# Autodesk Inventor assembly: meccanum_wheel_base_norm
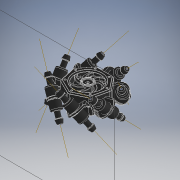
[picture p0: Inventor's stored thumbnail of the model, 180x180]
Saved by Autodesk Inventor 2022 (Build 260153000, 153)
## iProperties
Created: 2023-01-06
Part Number: meccanum_wheel_base_norm
Document SubType Name: Assembly
Designer: Иван Петров
Author: Иван Петров
## Documents named in this file (3)
- C:\Users\Ivan Petrov\Documents\GitHub\OmniBot\design\standart_components\VEX Meccanum wheel\meccanum_wheel_base_norm.iam
- C:\Users\Ivan Petrov\Documents\GitHub\OmniBot\design\standart_components\VEX Meccanum wheel\meccanum_wheel_base.ipt
- C:\Users\Ivan Petrov\Documents\GitHub\OmniBot\design\standart_components\VEX Meccanum wheel\roller_as,.iam
## Components (2 placed, 2 different names)
1. meccanum_wheel_base:1 — Совмещение:1, Совмещение:2, Заподлицо:1, Совмещение:3, Совмещение:4, Совмещение:5, Заподлицо:2, Угол:1, Совмещение:6, Совмещение:7, Совмещение:8, Совмещение:9, Совмещение:10, Совмещение:11, Совмещение:12
2. roller_as,:1 [sub-assembly] — Совмещение:5, Заподлицо:2
## Relationships (15: Mate 12, Flush 2, Angle 1)
- Совмещение:1 [Mate]: meccanum_wheel_base:1
- Совмещение:2 [Mate]: meccanum_wheel_base:1
- Заподлицо:1 [Flush] (-1 mm): meccanum_wheel_base:1
- Совмещение:3 [Mate]: meccanum_wheel_base:1
- Совмещение:4 [Mate]: meccanum_wheel_base:1
- Совмещение:5 [Mate]: meccanum_wheel_base:1 ↔ roller_as,:1
- Заподлицо:2 [Flush]: meccanum_wheel_base:1 ↔ roller_as,:1
- Угол:1 [Angle] (0 deg): meccanum_wheel_base:1
- Совмещение:6 [Mate]: meccanum_wheel_base:1
- Совмещение:7 [Mate]: meccanum_wheel_base:1
- Совмещение:8 [Mate]: meccanum_wheel_base:1
- Совмещение:9 [Mate]: meccanum_wheel_base:1
- Совмещение:10 [Mate]: meccanum_wheel_base:1
- Совмещение:11 [Mate]: meccanum_wheel_base:1
- Совмещение:12 [Mate]: meccanum_wheel_base:1
